# Autodesk Inventor assembly: full_model_asm
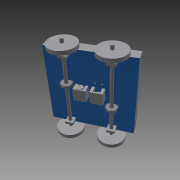
[picture p0: Inventor's stored thumbnail of the model, 180x180]
Saved by Autodesk Inventor 2015 (Build 190159000, 159)
## iProperties
Created: 2015-06-17
Part Number: full_model_asm
Document SubType Name: Assembly
Designer: Abhishyant
Author: Abhishyant
## Documents named in this file (6)
- D:\Projects\Personal\BroBot\3D Model\full_model_asm.iam
- D:\Projects\Personal\BroBot\3D Model\Body.ipt
- D:\Projects\Personal\BroBot\3D Model\Axle.ipt
- D:\Projects\Personal\BroBot\3D Model\Wheel.ipt
- D:\Projects\Personal\BroBot\3D Model\dc_motor.ipt
- D:\Projects\Personal\BroBot\3D Model\axle_gear.iam
## Components (11 placed, 5 different names)
1. Body:1 — back_axle, front_axle, Mate:1, Mate:2
2. Axle:1 — front_axle, front_left_wheel, front_right_wheel, Cylindrical:7
3. Axle:2 — back_axle, back_left_wheel, back_right_wheel, Cylindrical:8
4. Wheel:1 — back_left_wheel
5. Wheel:2 — front_right_wheel
6. Wheel:3 — back_right_wheel
7. Wheel:4 — front_left_wheel
8. dc_motor:1 — Mate:2
9. dc_motor:2 — Mate:1
10. axle_gear:1 [sub-assembly] — Cylindrical:7
11. axle_gear:2 [sub-assembly] — Cylindrical:8
## Relationships (10: CylindricalJoint 8, Mate 2)
- back_axle [CylindricalJoint]: Body:1 ↔ Axle:2
- front_axle [CylindricalJoint]: Body:1 ↔ Axle:1
- front_left_wheel [CylindricalJoint]: Axle:1 ↔ Wheel:4
- back_left_wheel [CylindricalJoint]: Axle:2 ↔ Wheel:1
- front_right_wheel [CylindricalJoint]: Axle:1 ↔ Wheel:2
- back_right_wheel [CylindricalJoint]: Axle:2 ↔ Wheel:3
- Mate:1 (15 mm): Body:1 ↔ dc_motor:2
- Mate:2 (15 mm): Body:1 ↔ dc_motor:1
- Cylindrical:7: Axle:1 ↔ axle_gear:1
- Cylindrical:8: Axle:2 ↔ axle_gear:2
